# Autodesk Inventor assembly: FinalExtruder
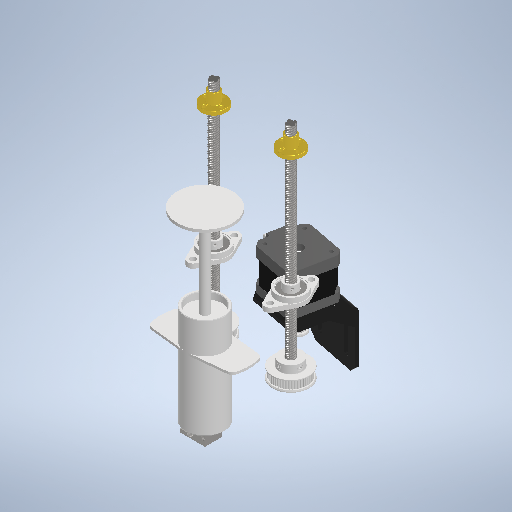
[picture p0: Inventor's stored thumbnail of the model, 512x512]
Saved by Autodesk Inventor 2025.2 (Build 292293000, 293)
## iProperties
Created: 2025-06-23
Part Number: FinalExtruder
Document SubType Name: Assembly
Designer: Simon
Author: Simon
## Documents named in this file (12)
- C:\Users\Simon\OneDrive\Documents\Inventor\Skripsie2025\Final System\Final Extruder\FinalExtruder.iam
- C:\Users\Simon\OneDrive\Documents\Inventor\Skripsie2025\PartsFolder\0.4 nozzle.ipt
- C:\Users\Simon\OneDrive\Documents\Inventor\Skripsie2025\PartsFolder\E3D-v6 Heater Block for Sensor Cartridges.ipt
- C:\Users\Simon\OneDrive\Documents\Inventor\Skripsie2025\Final System\Final Extruder\Plunger.ipt
- C:\Users\Simon\OneDrive\Documents\Inventor\Skripsie2025\Final System\Final Extruder\TR8x8-4_LeadScrew_200mm.ipt
- C:\Users\Simon\OneDrive\Documents\Inventor\Skripsie2025\Final System\Final Extruder\Cylinder.ipt
- C:\Users\Simon\OneDrive\Documents\Inventor\Skripsie2025\PartsFolder\Stepper_17HS4401.ipt
- C:\Users\Simon\OneDrive\Documents\Inventor\Skripsie2025\PartsFolder\TR8x8-4_Nut.ipt
- C:\Users\Simon\OneDrive\Documents\Inventor\Skripsie2025\PartsFolder\GT2_16T Pulley.ipt
- C:\Users\Simon\OneDrive\Documents\Inventor\Skripsie2025\PartsFolder\GT2_48T_8.ipt
- C:\Users\Simon\OneDrive\Documents\Inventor\Skripsie2025\PartsFolder\Pillow Block Bearing 1\Zinc Alloy Pillow Block Flange Bearing KFL08 ID-8mm.iam
- C:\Users\Simon\OneDrive\Documents\Inventor\Skripsie2025\PartsFolder\bracket nema 17.ipt
## Components (15 placed, 11 different names)
1. 0.4 nozzle:1 — Mate:1, Mate:2, Angle:1
2. E3D-v6 Heater Block for Sensor Cartridges:1 — Mate:1, Mate:2, Angle:1, Mate:3, Mate:4
3. Plunger:1 — Mate:5
4. TR8x8-4_LeadScrew_200mm:1 — Mate:7, Mate:9, Mate:11, Flush:2
5. TR8x8-4_LeadScrew_200mm:2 — Mate:6, Mate:8, Mate:12, Flush:1
6. Cylinder:1 — Mate:3, Mate:4, Mate:5
7. Stepper_17HS4401:1 — Mate:10, Mate:13, Angle:2, Flush:6
8. TR8x8-4_Nut:1 — Mate:6
9. TR8x8-4_Nut:2 — Mate:7
10. GT2_16T Pulley:1 — Mate:10, Flush:5, Flush:6
11. GT2_48T_8:1 — Mate:9, Flush:2, Flush:3, Flush:5
12. GT2_48T_8:2 — Mate:8, Flush:1, Flush:3
13. Zinc Alloy Pillow Block Flange Bearing KFL08 ID-8mm:1 [sub-assembly] — Mate:11, Flush:4
14. Zinc Alloy Pillow Block Flange Bearing KFL08 ID-8mm:2 [sub-assembly] — Mate:12, Flush:4
15. bracket nema 17:1 — Mate:13, Angle:2
## Relationships (21: Mate 13, Flush 6, Angle 2)
- Mate:1: 0.4 nozzle:1 ↔ E3D-v6 Heater Block for Sensor Cartridges:1
- Mate:2: 0.4 nozzle:1 ↔ E3D-v6 Heater Block for Sensor Cartridges:1
- Angle:1 (0 deg): 0.4 nozzle:1 ↔ E3D-v6 Heater Block for Sensor Cartridges:1
- Mate:3: E3D-v6 Heater Block for Sensor Cartridges:1 ↔ Cylinder:1
- Mate:4: E3D-v6 Heater Block for Sensor Cartridges:1 ↔ Cylinder:1
- Mate:5: Plunger:1 ↔ Cylinder:1
- Mate:6: TR8x8-4_LeadScrew_200mm:2 ↔ TR8x8-4_Nut:1
- Mate:7: TR8x8-4_LeadScrew_200mm:1 ↔ TR8x8-4_Nut:2
- Mate:8: TR8x8-4_LeadScrew_200mm:2 ↔ GT2_48T_8:2
- Mate:9: TR8x8-4_LeadScrew_200mm:1 ↔ GT2_48T_8:1
- Mate:10: Stepper_17HS4401:1 ↔ GT2_16T Pulley:1
- Mate:11: TR8x8-4_LeadScrew_200mm:1 ↔ Zinc Alloy Pillow Block Flange Bearing KFL08 ID-8mm:1
- Mate:12: TR8x8-4_LeadScrew_200mm:2 ↔ Zinc Alloy Pillow Block Flange Bearing KFL08 ID-8mm:2
- Flush:1: TR8x8-4_LeadScrew_200mm:2 ↔ GT2_48T_8:2
- Flush:2: TR8x8-4_LeadScrew_200mm:1 ↔ GT2_48T_8:1
- Flush:3: GT2_48T_8:1 ↔ GT2_48T_8:2
- Flush:4: Zinc Alloy Pillow Block Flange Bearing KFL08 ID-8mm:1 ↔ Zinc Alloy Pillow Block Flange Bearing KFL08 ID-8mm:2
- Flush:5: GT2_16T Pulley:1 ↔ GT2_48T_8:1
- Mate:13: Stepper_17HS4401:1 ↔ bracket nema 17:1
- Angle:2 (0 deg): Stepper_17HS4401:1 ↔ bracket nema 17:1
- Flush:6 (-5 mm): Stepper_17HS4401:1 ↔ GT2_16T Pulley:1
